# Autodesk Inventor assembly: Gancho
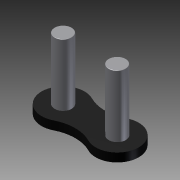
[picture p0: Inventor's stored thumbnail of the model, 180x180]
Saved by Autodesk Inventor 2011 (Build 150239000, 239)
## iProperties
Created: 2011-08-31
Part Number: Gancho
Document SubType Name: Assembly
Designer: Luis
Author: Luis
## Documents named in this file (3)
- C:\Documents and Settings\Luis\Mis documentos\Inventor\Cadena 428\Gancho.iam
- C:\Documents and Settings\Luis\Mis documentos\Inventor\Cadena 428\Concha1.ipt
- C:\Documents and Settings\Luis\Mis documentos\Inventor\Cadena 428\Pasador.ipt
## Components (3 placed, 2 different names)
1. Concha1:1 — Insert:1, Insert:2
2. Pasador:1 — Insert:1
3. Pasador:2 — Insert:2
## Relationships (2: Insert 2)
- Insert:1 (-0.5 mm): Concha1:1 ↔ Pasador:1
- Insert:2 (-0.5 mm): Concha1:1 ↔ Pasador:2
